# Autodesk Inventor assembly: mid_heater_assemble
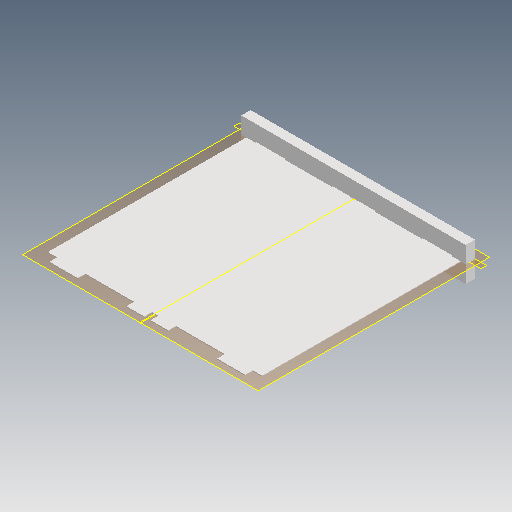
[picture p0: Inventor's stored thumbnail of the model, 512x512]
Saved by Autodesk Inventor 2020 (Build 240168000, 168)
## iProperties
Created: 2021-05-08
Part Number: mid_heater_assemble
Document SubType Name: Assembly
Designer: Hsu Daniel
Author: Hsu Daniel
## Documents named in this file (3)
- D:\Daniel\NTU\makeNTU2021\大改\mid_heater_assemble.iam
- D:\Daniel\NTU\makeNTU2021\大改\mid_heater.ipt
- D:\Daniel\NTU\makeNTU2021\大改\mid_bottom.ipt
## Components (2 placed, 2 different names)
1. mid_heater:1 — Flush:1, Flush:2, Mate:1
2. mid_bottom:1 — Flush:1, Flush:2, Mate:1
## Relationships (3: Flush 2, Mate 1)
- Flush:1: mid_heater:1 ↔ mid_bottom:1
- Flush:2: mid_heater:1 ↔ mid_bottom:1
- Mate:1: mid_heater:1 ↔ mid_bottom:1
